# Autodesk Inventor assembly: leg
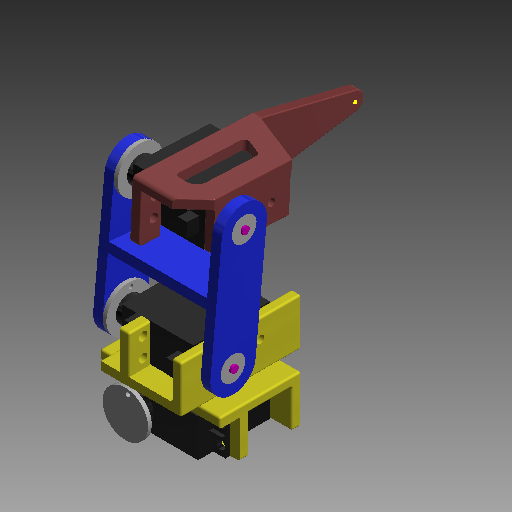
[picture p0: Inventor's stored thumbnail of the model, 512x512]
Saved by Autodesk Inventor 2017 (Build 210142000, 142)
## iProperties
Part Number: leg
Document SubType Name: Assembly
Designer: Alexander Miller
Author: Alexander Miller
## Documents named in this file (7)
- D:\Daten\Documents\Git\Hexapod\3DParts\leg_right.iam
- D:\Daten\Documents\Git\Hexapod\3DParts\Serov_with_arm.iam
- D:\Daten\Documents\Git\Hexapod\3DParts\Upper_leg.ipt
- D:\Daten\Documents\Git\Hexapod\3DParts\Middle_leg.ipt
- D:\Daten\Documents\Git\Hexapod\3DParts\ball_bearing.ipt
- D:\Daten\Documents\Git\Hexapod\3DParts\Lower_leg_right.ipt
- D:\Daten\Documents\Git\Hexapod\3DParts\Connector.ipt
## Components (11 placed, 6 different names)
1. Serov_with_arm:1 [sub-assembly] — Rigid:17, Rigid:20
2. Serov_with_arm:2 [sub-assembly] — Rigid:8
3. Upper_leg:1 — Rigid:14, Rigid:20, Rigid:21
4. Upper_leg:2 — Rigid:8, Rigid:14
5. Middle_leg:1 — Rigid:15, Rigid:16, Rigid:17, Rigid:18
6. Serov_with_arm:3 [sub-assembly] — Rigid:18, Rigid:19
7. ball_bearing:1 — Rigid:15
8. ball_bearing:2 — Rigid:16
9. Lower_leg_right:1 — Rigid:19, Rigid:22
10. Connector:1 — Rigid:22
11. Connector:2 — Rigid:21
## Relationships (10: WeldJoint 10)
- Rigid:8 [WeldJoint]: Serov_with_arm:2 ↔ Upper_leg:2
- Rigid:14 [WeldJoint]: Upper_leg:1 ↔ Upper_leg:2
- Rigid:15 [WeldJoint]: Middle_leg:1 ↔ ball_bearing:1
- Rigid:16 [WeldJoint]: Middle_leg:1 ↔ ball_bearing:2
- Rigid:17 [WeldJoint]: Serov_with_arm:1 ↔ Middle_leg:1
- Rigid:18 [WeldJoint]: Middle_leg:1 ↔ Serov_with_arm:3
- Rigid:19 [WeldJoint]: Serov_with_arm:3 ↔ Lower_leg_right:1
- Rigid:20 [WeldJoint]: Serov_with_arm:1 ↔ Upper_leg:1
- Rigid:21 [WeldJoint]: Upper_leg:1 ↔ Connector:2
- Rigid:22 [WeldJoint]: Lower_leg_right:1 ↔ Connector:1
